# Autodesk Inventor assembly: Top_Assembly_4axis
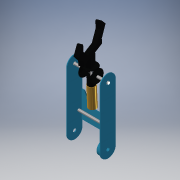
[picture p0: Inventor's stored thumbnail of the model, 180x180]
Saved by Autodesk Inventor 2016 (Build 200138000, 138)
## iProperties
Created: 2015-05-21
Part Number: Top_Assembly_4axis
Document SubType Name: Assembly
Designer: CHUNGBK
Author: CHUNGBK
## Documents named in this file (6)
- C:\Users\jonathan\Desktop\Five Axis Serial Robotic Arm\Inventor\Scorbot Gripper.iam
- C:\Users\jonathan\Desktop\Five Axis Serial Robotic Arm\Inventor\Scorbot Elbow.iam
- C:\Users\jonathan\Desktop\Five Axis Serial Robotic Arm\Inventor\Gripper Motor.ipt
- C:\Users\jonathan\Desktop\Five Axis Serial Robotic Arm\Inventor\Bevel Gear.ipt
- C:\Users\jonathan\Desktop\Five Axis Serial Robotic Arm\Inventor\Gripper Gear.ipt
- C:\Users\jonathan\Desktop\Five Axis Serial Robotic Arm\Inventor\Motor Shaft.ipt
## Components (6 placed, 4 different names)
1. Scorbot Elbow:1 [sub-assembly] — Flush:1, Flush:2, Flush:3, Mate:1, Mate:2, Mate:3, Mate:4, Mate:10, Mate:11
2. Gripper Motor:1 — Mate:5, Mate:6, Mate:10
3. Bevel Gear1:1 — Mate:1, Mate:2
4. Bevel Gear1:2 — Mate:3, Mate:4
5. Bevel Gear1:3 — Mate:7, Mate:8, Mate:11
6. Motor Shaft:1 — Mate:5, Mate:6, Mate:7, Mate:8
## Relationships (13: Mate 10, Flush 3)
- Flush:1: Scorbot Elbow:1
- Flush:2: Scorbot Elbow:1
- Flush:3: Scorbot Elbow:1
- Mate:1: Scorbot Elbow:1 ↔ Bevel Gear1:1
- Mate:2: Scorbot Elbow:1 ↔ Bevel Gear1:1
- Mate:3: Scorbot Elbow:1 ↔ Bevel Gear1:2
- Mate:4: Scorbot Elbow:1 ↔ Bevel Gear1:2
- Mate:5: Gripper Motor:1 ↔ Motor Shaft:1
- Mate:6: Gripper Motor:1 ↔ Motor Shaft:1
- Mate:7: Bevel Gear1:3 ↔ Motor Shaft:1
- Mate:8: Bevel Gear1:3 ↔ Motor Shaft:1
- Mate:10 (61.9125 mm): Scorbot Elbow:1 ↔ Gripper Motor:1
- Mate:11: Scorbot Elbow:1 ↔ Bevel Gear1:3
